# Autodesk Inventor assembly: #Spindexer
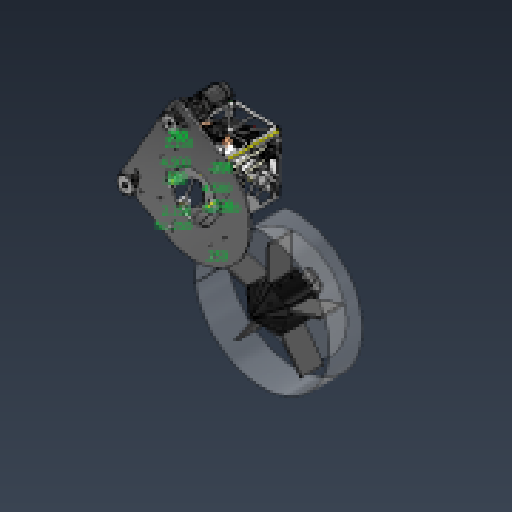
[picture p0: Inventor's stored thumbnail of the model, 512x512]
Saved by Autodesk Inventor 2026 (Build 300175050, 175E)
## iProperties
Created: 2026-02-05
Part Number: #Spindexer
Document SubType Name: Assembly
Designer: Owen L
Mass: 7775.4 g
Surface Area: 19734.6 cm^2
Volume: 5821.17 cm^3
Density: 1.33571 g/cm^3
Author: Owen L
## Documents named in this file (49)
- C:\Users\Jthib\Documents\GitHub\2026-Robot-Mechanical\Spindexer\#Spindexer.iam
- C:\Users\Jthib\Documents\GitHub\2026-Robot-Mechanical\Spindexer\3DPRINT,HUB.ipt
- C:\Users\Jthib\Documents\GitHub\2026-Robot-Mechanical\Spindexer\3DPRINT,HUB,CONE.ipt
- C:\Users\Jthib\Documents\GitHub\2026-Robot-Mechanical\Spindexer\PLATE,WALL.ipt
- C:\Users\Jthib\Documents\GitHub\2026-Robot-Mechanical\Spindexer\PLATE,BOTTOM.ipt
- C:\Users\Jthib\Documents\GitHub\2026-Robot-Mechanical\Spindexer\STOCK,HEX,SHAFT,HUB.ipt
- C:\Users\Jthib\Documents\GitHub\2026-Robot-Mechanical\Spindexer\PLATE,KICKER,OUTSIDE.ipt
- C:\Users\Jthib\Documents\GitHub\2026-Robot-Mechanical\Spindexer\3DPRINT,KICKER,RAMP.ipt
- C:\Users\Jthib\Documents\GitHub\2026-Robot-Mechanical\Spindexer\PLATE,KICKER,INSIDE.ipt
- C:\Users\Jthib\Documents\GitHub\2026-Robot-Mechanical\Spindexer\STOCK,HEX,SHAFT,KICKER,FRONT.ipt
- C:\Users\Jthib\Documents\GitHub\2026-Robot-Mechanical\Spindexer\STOCK,HEX,SHAFT,KICKER,BACK.ipt
- C:\Users\Jthib\Documents\GitHub\2026-Robot-Mechanical\#1_CAD Library\Power Transmission\Bearings\PURCHASED,HEX_BEARING.ipt
- C:\Users\Jthib\Documents\GitHub\2026-Robot-Mechanical\#1_CAD Library\Power Transmission\VersaPlanetary\GEARBOX,VERSAPLANETARY,SINGLE-STAGE,HEX-SHAFT,0.5IN.ipt
- C:\Users\Jthib\Documents\GitHub\2026-Robot-Mechanical\#1_CAD Library\Power Transmission\VersaPlanetary\ADAPTER,CIM-NEO,VERSAPLANETARY.ipt
- C:\Users\Jthib\Documents\GitHub\2026-Robot-Mechanical\#1_CAD Library\Motors\MOTOR,REV,NEO,V1-1.ipt
- C:\Users\Jthib\Documents\GitHub\2026-Robot-Mechanical\Spindexer\PLATE,NUT-BLOCK,3-LONG.ipt
- C:\Users\Jthib\Documents\GitHub\2026-Robot-Mechanical\Spindexer\PLATE,NUT-BLOCK,2-LONG.ipt
- C:\Users\Jthib\Documents\GitHub\2026-Robot-Mechanical\Spindexer\PLATE,NUT-BLOCK,1-LONG.ipt
- C:\Users\Jthib\Documents\GitHub\2026-Robot-Mechanical\#1_CAD Library\Electronics\CONTROLS,SPARK_MAX.ipt
- C:\Users\Jthib\Documents\GitHub\2026-Robot-Mechanical\Spindexer\3DPRINT,SPARK_MAX,MOUNT.ipt
- C:\Users\Jthib\Documents\GitHub\2026-Robot-Mechanical\Spindexer\PLATE,KICKER,BACK.ipt
- C:\Users\Jthib\Documents\GitHub\2026-Robot-Mechanical\Spindexer\PLATE,NUT-BLOCK,L-SHAPE.ipt
- C:\Users\Jthib\Documents\GitHub\2026-Robot-Mechanical\Spindexer\3DPRINTED,PULLEY,21T,9mm.ipt
- C:\Users\Jthib\Documents\GitHub\2026-Robot-Mechanical\#1_CAD Library\Power Transmission\Pulleys\PURCHASED,HTD5mm,24T,PULLEY.ipt
- C:\Users\Jthib\Documents\GitHub\2026-Robot-Mechanical\Spindexer\STANDIN,BELT,70T,HTD5mm.ipt
- C:\Users\Jthib\Documents\GitHub\2026-Robot-Mechanical\Spindexer\STANDIN,BELT,100T,HTD5mm.ipt
- C:\Users\Jthib\Documents\GitHub\2026-Robot-Mechanical\#1_CAD Library\Building Materials\Fasteners\Bolts\PURCHASED,10-32x0.5in,BUTTONHEAD,BOLT.ipt
- C:\Users\Jthib\Documents\GitHub\2026-Robot-Mechanical\#1_CAD Library\Building Materials\Fasteners\Nuts\PURCHASED,NYLOCK,10-32,NUT.ipt
- C:\Users\Jthib\Documents\GitHub\2026-Robot-Mechanical\#1_CAD Library\Building Materials\Fasteners\Bolts\PURCHASED,10-32x0.625in,BUTTONHEAD,BOLT.ipt
- C:\Users\Jthib\Documents\GitHub\2026-Robot-Mechanical\Spindexer\PLATE,NUT-BLOCK,SINGLE-L.ipt
- C:\Users\Jthib\Documents\GitHub\2026-Robot-Mechanical\Spindexer\PLATE,SHOOTER,MOUNT.ipt
- C:\Users\Jthib\Documents\GitHub\2026-Robot-Mechanical\Spindexer\#Spindexer\Design Accelerator\PLATE,TURRET,ENCODER,GEAR.ipt
- C:\Users\Jthib\Documents\GitHub\2026-Robot-Mechanical\Spindexer\#Spindexer\Design Accelerator\PLATE,TURRET,PINNION,GEAR.ipt
- C:\Users\Jthib\Documents\GitHub\2026-Robot-Mechanical\Spindexer\#Spindexer\Design Accelerator\PLATE,TURRET,MOTOR,MOUNT.ipt
- C:\Users\Jthib\Documents\GitHub\2026-Robot-Mechanical\#1_CAD Library\Electronics\CONTROLS,ENCODER,HEX_BORE.ipt
- C:\Users\Jthib\Documents\GitHub\2026-Robot-Mechanical\Spindexer\#Spindexer\Design Accelerator\STOCK,HEX,SHAFT,TURRET,DRIVE.ipt
- C:\Users\Jthib\Documents\GitHub\2026-Robot-Mechanical\Spindexer\#Spindexer\Design Accelerator\STOCK,HEX,SHAFT,TURRET,ENCODER.ipt
- C:\Users\Jthib\Documents\GitHub\2026-Robot-Mechanical\Spindexer\#Spindexer\Design Accelerator\3DPRINT,TURRET,HEX,SPACER.ipt
- C:\Users\Jthib\Documents\GitHub\2026-Robot-Mechanical\Spindexer\STOCK,CHURRO,HEX,TURRET,MOTOR-MOUNT,SPACER.ipt
- C:\Users\Jthib\Documents\GitHub\2026-Robot-Mechanical\#1_CAD Library\Building Materials\Fasteners\Bolts\PURCHASED,0.25-20x0.5in,BUTTONHEAD,BOLT.ipt
- C:\Users\Jthib\Documents\GitHub\2026-Robot-Mechanical\Spindexer\3DRPINT,FRONT-ROLLER,DRIVE-SPACER.ipt
- C:\Users\Jthib\Documents\GitHub\2026-Robot-Mechanical\Spindexer\CAST,SLAB-OF-FLOP.ipt
- C:\Users\Jthib\Documents\GitHub\2026-Robot-Mechanical\Spindexer\PURCHASED,20-1,90deg,MAX-PLANETARY.ipt
- C:\Users\Jthib\Documents\GitHub\2026-Robot-Mechanical\#1_CAD Library\Motors\MOTOR,NEO,V2.0.ipt
- C:\Users\Jthib\Documents\GitHub\2026-Robot-Mechanical\#1_CAD Library\Wheels\Compliant\PURCHASED,WHEEL,COMPLIANT,2.25in.ipt
- C:\Users\Jthib\Documents\GitHub\2026-Robot-Mechanical\Spindexer\MOTOR,VEX,FALCON,500.ipt
- C:\Users\Jthib\Documents\GitHub\2026-Robot-Mechanical\#1_CAD Library\Power Transmission\MaxPlanetary\PURCHASED,REV,MAX-PLANETARY,SINGLE-STAGE,FALCON-TO-HEX.ipt
- C:\Users\Jthib\Documents\GitHub\2026-Robot-Mechanical\#1_CAD Library\Building Materials\Fasteners\Bolts\PURCHASED,10-32x0.625in,FLATHEAD,BOLT.ipt
- C:\Users\Jthib\Documents\GitHub\2026-Robot-Mechanical\#1_CAD Library\Building Materials\Fasteners\Washers\PURCHASED,WASHER,10-32.ipt
## Components (176 placed, 48 different names)
1. 3DPRINT,HUB:1 — Mate:11, Mate:12, Mate:13, Mate:15, Mate:16, Mate:17, Flush:2, Mate:106, Mate:107, Mate:108, Mate:109, Mate:110, Mate:111, Mate:112, Mate:113, Mate:114, Mate:117, Mate:118, Mate:119, Mate:120
2. 3DPRINT,HUB,CONE:1 — Mate:11, Mate:12, Mate:13
3. PLATE,WALL:1 — Flush:8, Mate:42, Mate:43, Flush:24
4. PLATE,BOTTOM:1 — Mate:117, Mate:118, Mate:119, Flush:24, Mate:122
5. STOCK,HEX,SHAFT,HUB:1 — Mate:16, Mate:17, Flush:2, Mate:121
6. PLATE,KICKER,OUTSIDE:1 — Mate:22, Mate:23, Mate:24, Mate:25, Flush:3, Flush:4, Flush:8, Insert:1, Insert:4, Mate:34, Mate:35, Mate:42, Insert:9, Insert:10, Insert:13, Flush:12, Mate:43, Insert:23, Insert:24, Insert:34, Insert:35, Insert:39, Insert:40, Insert:41, Insert:42, Insert:43, Insert:44, Insert:45, Insert:46, Insert:47, Insert:48, Insert:49, Insert:50, Insert:79, Insert:80, Insert:81, Insert:82, Mate:59, Insert:83, Mate:62, Insert:87, Insert:93, Insert:94, Mate:65, Mate:138, Mate:139, Insert:213, Insert:214
7. 3DPRINT,KICKER,RAMP:1 — Mate:22, Mate:23, Mate:24
8. PLATE,KICKER,INSIDE:1 — Mate:25, Flush:3, Flush:4, Insert:2, Insert:3, Mate:39, Mate:40, Mate:41, Insert:14, Insert:21, Insert:22, Insert:31, Insert:32, Insert:33, Mate:48, Mate:52, Insert:61, Insert:65, Insert:66, Insert:67, Insert:68, Insert:69, Insert:70, Insert:71, Insert:72, Insert:73, Insert:74, Insert:75, Insert:76, Insert:77, Insert:78, Mate:60, Insert:84, Mate:61, Insert:90, Insert:210, Insert:211, Insert:212
9. STOCK,HEX,SHAFT,KICKER,FRONT:1 — Mate:34, Mate:45, Flush:15, Mate:128, Mate:129, Mate:130
10. STOCK,HEX,SHAFT,KICKER,BACK:1 — Mate:35, Mate:46, Mate:47, Flush:14, Mate:131, Mate:132, Mate:133
11. PURCHASED,HEX_BEARING:1 — Insert:1, Flush:15
12. PURCHASED,HEX_BEARING:2 — Insert:2, Mate:103, Mate:104
13. PURCHASED,HEX_BEARING:3 — Insert:3, Mate:63
14. PURCHASED,HEX_BEARING:4 — Insert:4, Flush:14
15. GEARBOX,VERSAPLANETARY,SINGLE-STAGE,HEX-SHAFT,0.5IN:1 — Mate:36, Mate:37, Mate:38, Mate:39, Mate:40, Mate:41, Mate:53
16. ADAPTER,CIM-NEO,VERSAPLANETARY:1 — Mate:36, Mate:37, Mate:38, Insert:5
17. MOTOR,REV,NEO,V1-1:1 — Insert:5
18. PLATE,NUT-BLOCK,3-LONG:1 — Mate:60, Insert:84
19. PLATE,NUT-BLOCK,3-LONG:2 — Insert:9, Insert:10
20. PLATE,NUT-BLOCK,3-LONG:3 — Mate:59, Insert:83
21. PLATE,NUT-BLOCK,1-LONG:1 — Insert:13, Flush:11, Flush:12
22. PLATE,NUT-BLOCK,1-LONG:2 — Insert:14, Flush:11
23. PLATE,NUT-BLOCK,3-LONG:4 — Mate:66, Insert:210
24. PLATE,NUT-BLOCK,3-LONG:5 — Insert:93, Insert:94, Mate:67
25. CONTROLS,SPARK_MAX:1 — Mate:125, Mate:126, Mate:127
26. 3DPRINT,SPARK_MAX,MOUNT:1 — Insert:149, Mate:124, Mate:126, Mate:127
27. PLATE,KICKER,BACK:1 — Mate:44, Insert:25, Insert:26, Insert:27, Insert:28, Insert:51, Insert:52, Insert:53, Insert:54, Insert:55, Insert:59, Insert:60, Insert:85, Insert:86, Insert:88, Insert:89, Insert:149, Mate:124, Mate:125, Insert:229, Insert:230
28. PLATE,NUT-BLOCK,2-LONG:2 — Insert:21, Insert:22, Mate:44, Insert:26
29. PLATE,NUT-BLOCK,2-LONG:3 — Insert:23, Insert:24, Insert:25
30. PLATE,NUT-BLOCK,3-LONG:6 — Insert:27, Insert:28
31. PLATE,NUT-BLOCK,3-LONG:8 — Insert:31, Insert:32
32. PLATE,NUT-BLOCK,L-SHAPE:1 — Insert:33
33. PLATE,NUT-BLOCK,L-SHAPE:2 — Insert:34
34. 3DPRINTED,PULLEY,21T,9mm:1 — Mate:46, Mate:55, Mate:58, Mate:64, Flush:16
35. 3DPRINTED,PULLEY,21T,9mm:2 — Mate:45, Mate:54, Flush:16
36. PURCHASED,HEX_BEARING:5 — Mate:52, Mate:53
37. PURCHASED,HTD5mm,24T,PULLEY:1 — Mate:47, Flush:13, Mate:57, Mate:63, Mate:64
38. PURCHASED,HTD5mm,24T,PULLEY:2 — Mate:48, Flush:13, Mate:56
39. STANDIN,BELT,70T,HTD5mm:1 — Mate:56, Mate:57
40. STANDIN,BELT,100T,HTD5mm:1 — Mate:54, Mate:55, Mate:58
41. PURCHASED,10-32x0.5in,BUTTONHEAD,BOLT:1 — Insert:48
42. PURCHASED,NYLOCK,10-32,NUT:1 — Insert:81
43. PURCHASED,10-32x0.625in,BUTTONHEAD,BOLT:1 — Insert:35
44. PURCHASED,10-32x0.625in,BUTTONHEAD,BOLT:5 — Insert:39
45. PURCHASED,10-32x0.625in,BUTTONHEAD,BOLT:6 — Insert:40
46. PURCHASED,10-32x0.625in,BUTTONHEAD,BOLT:7 — Insert:41
47. PURCHASED,10-32x0.625in,BUTTONHEAD,BOLT:8 — Insert:42
48. PURCHASED,10-32x0.625in,BUTTONHEAD,BOLT:9 — Insert:43
49. PURCHASED,10-32x0.625in,BUTTONHEAD,BOLT:10 — Insert:44
50. PURCHASED,10-32x0.625in,BUTTONHEAD,BOLT:11 — Insert:45
51. PURCHASED,10-32x0.625in,BUTTONHEAD,BOLT:12 — Insert:46
52. PURCHASED,10-32x0.625in,BUTTONHEAD,BOLT:13 — Insert:47
53. PURCHASED,10-32x0.625in,BUTTONHEAD,BOLT:14 — Insert:51
54. PURCHASED,10-32x0.625in,BUTTONHEAD,BOLT:15 — Insert:52
55. PURCHASED,10-32x0.625in,BUTTONHEAD,BOLT:16 — Insert:53
56. PURCHASED,10-32x0.625in,BUTTONHEAD,BOLT:17 — Insert:54
57. PURCHASED,10-32x0.625in,BUTTONHEAD,BOLT:18 — Insert:55
58. PURCHASED,10-32x0.5in,BUTTONHEAD,BOLT:2 — Insert:49
59. PURCHASED,10-32x0.5in,BUTTONHEAD,BOLT:3 — Insert:50
60. PURCHASED,10-32x0.625in,BUTTONHEAD,BOLT:19 — Insert:59
61. PURCHASED,10-32x0.625in,BUTTONHEAD,BOLT:20 — Insert:89
62. PURCHASED,10-32x0.625in,BUTTONHEAD,BOLT:21 — Insert:87
63. PURCHASED,10-32x0.625in,BUTTONHEAD,BOLT:22 — Insert:60
64. PURCHASED,10-32x0.625in,BUTTONHEAD,BOLT:23 — Insert:88
65. PURCHASED,10-32x0.625in,BUTTONHEAD,BOLT:24 — Insert:61
66. PURCHASED,10-32x0.625in,BUTTONHEAD,BOLT:28 — Insert:65
67. PURCHASED,10-32x0.625in,BUTTONHEAD,BOLT:29 — Insert:66
68. PURCHASED,10-32x0.625in,BUTTONHEAD,BOLT:30 — Insert:67
69. PURCHASED,10-32x0.625in,BUTTONHEAD,BOLT:31 — Insert:68
70. PURCHASED,10-32x0.625in,BUTTONHEAD,BOLT:32 — Insert:69
71. PURCHASED,10-32x0.625in,BUTTONHEAD,BOLT:33 — Insert:70
72. PURCHASED,10-32x0.625in,BUTTONHEAD,BOLT:34 — Insert:73
73. PURCHASED,10-32x0.625in,BUTTONHEAD,BOLT:35 — Insert:72
74. PURCHASED,10-32x0.625in,BUTTONHEAD,BOLT:36 — Insert:71
75. PURCHASED,10-32x0.5in,BUTTONHEAD,BOLT:4 — Insert:74
76. PURCHASED,10-32x0.5in,BUTTONHEAD,BOLT:5 — Insert:76
77. PURCHASED,10-32x0.5in,BUTTONHEAD,BOLT:6 — Insert:75
78. PURCHASED,10-32x0.5in,BUTTONHEAD,BOLT:7 — Insert:77
79. PURCHASED,10-32x0.5in,BUTTONHEAD,BOLT:8 — Insert:78
80. PURCHASED,10-32x0.5in,BUTTONHEAD,BOLT:9 — Insert:79
81. PURCHASED,10-32x0.5in,BUTTONHEAD,BOLT:10 — Insert:80
82. PURCHASED,NYLOCK,10-32,NUT:2 — Insert:82
83. PLATE,NUT-BLOCK,SINGLE-L:1 — Insert:85, Mate:61
84. PLATE,NUT-BLOCK,SINGLE-L:2 — Insert:86, Mate:62
85. PURCHASED,10-32x0.625in,BUTTONHEAD,BOLT:37 — Insert:90
86. PLATE,SHOOTER,MOUNT:1 — Mate:65, Mate:66, Mate:67, Mate:82, Mate:95, Mate:100, Insert:142, Insert:143, Insert:144, Insert:145, Insert:146, Insert:147, Insert:150, Insert:151, Insert:152, Insert:153, Insert:154, Insert:158, Insert:159, Insert:160, Insert:164, Insert:165, Insert:166, Insert:168, Insert:169, Insert:170, Mate:150, Mate:151, Insert:185, Insert:186, Insert:187, Insert:188, Insert:221, Insert:222, Insert:223, Insert:224, Insert:225, Insert:226, Insert:227, Insert:228, Insert:231, Insert:233, Insert:235, Insert:237
87. PLATE,TURRET,ENCODER,GEAR:1 — Mate:102, Mate:143, Flush:26
88. PLATE,TURRET,PINNION,GEAR:1 — Mate:86, Flush:25, Mate:140, Mate:141
89. PURCHASED,HEX_BEARING:6 — Mate:83, Mate:86, Mate:93, Insert:154
90. PURCHASED,HEX_BEARING:7 — Mate:94, Mate:96, Insert:153, Mate:145
91. PLATE,TURRET,MOTOR,MOUNT:1 — Mate:100, Insert:155, Insert:156, Insert:157, Insert:161, Insert:162, Insert:163, Insert:174, Insert:175, Insert:176, Insert:177, Mate:147, Insert:178, Mate:148
92. CONTROLS,ENCODER,HEX_BORE:1 — Mate:95, Mate:96, Insert:236, Insert:238
93. CONTROLS,ENCODER,HEX_BORE:2 — Mate:82, Mate:83, Insert:232, Insert:234
94. STOCK,HEX,SHAFT,TURRET,DRIVE:1 — Flush:25, Mate:140, Mate:142, Insert:215
95. STOCK,HEX,SHAFT,TURRET,ENCODER:1 — Mate:143, Flush:26, Mate:144, Insert:216, Insert:217
96. 3DPRINT,TURRET,HEX,SPACER:1 — Mate:94, Mate:102, Mate:144, Mate:145
97. 3DPRINT,TURRET,HEX,SPACER:2 — Mate:93, Mate:141, Mate:142
98. PURCHASED,10-32x0.625in,BUTTONHEAD,BOLT:44 — Mate:150, Insert:231
99. PURCHASED,10-32x0.625in,BUTTONHEAD,BOLT:45 — Insert:233
100. PURCHASED,NYLOCK,10-32,NUT:5 — Insert:234
101. PURCHASED,NYLOCK,10-32,NUT:6 — Insert:232
102. STOCK,CHURRO,HEX,TURRET,MOTOR-MOUNT,SPACER:1 — Insert:150
103. STOCK,CHURRO,HEX,TURRET,MOTOR-MOUNT,SPACER:2 — Insert:152, Insert:157
104. STOCK,CHURRO,HEX,TURRET,MOTOR-MOUNT,SPACER:3 — Insert:151, Insert:156
105. STOCK,CHURRO,HEX,TURRET,MOTOR-MOUNT,SPACER:4 — Insert:164, Mate:146
106. PURCHASED,0.25-20x0.5in,BUTTONHEAD,BOLT:4 — Insert:158
107. 3DRPINT,FRONT-ROLLER,DRIVE-SPACER:1 — Mate:103, Mate:104
108. PURCHASED,10-32x0.625in,BUTTONHEAD,BOLT:46 — Mate:151, Insert:237
109. PURCHASED,10-32x0.625in,BUTTONHEAD,BOLT:47 — Insert:235
110. PURCHASED,NYLOCK,10-32,NUT:7 — Insert:238
111. PURCHASED,NYLOCK,10-32,NUT:8 — Insert:236
112. CAST,SLAB-OF-FLOP:1 — Mate:106, Mate:107
113. CAST,SLAB-OF-FLOP:2 — Mate:108, Mate:109
114. CAST,SLAB-OF-FLOP:3 — Mate:110, Mate:111
115. CAST,SLAB-OF-FLOP:4 — Mate:112, Mate:113
116. CAST,SLAB-OF-FLOP:5 — Mate:114, Mate:120
117. PURCHASED,10-32x0.625in,BUTTONHEAD,BOLT:52 — Insert:142
118. PURCHASED,10-32x0.625in,BUTTONHEAD,BOLT:53 — Insert:143
119. PURCHASED,10-32x0.625in,BUTTONHEAD,BOLT:54 — Insert:144
120. PURCHASED,10-32x0.625in,BUTTONHEAD,BOLT:55 — Insert:145
121. PURCHASED,10-32x0.625in,BUTTONHEAD,BOLT:56 — Insert:146
122. PURCHASED,10-32x0.625in,BUTTONHEAD,BOLT:57 — Insert:147
123. PURCHASED,20-1,90deg,MAX-PLANETARY:1 — Mate:121, Mate:122, Insert:148, Mate:123
124. MOTOR,NEO,V2.0:1 — Insert:148, Mate:123
125. PURCHASED,WHEEL,COMPLIANT,2.25in:1 — Mate:128, Mate:136, Mate:137
126. PURCHASED,WHEEL,COMPLIANT,2.25in:2 — Mate:129, Mate:137
127. PURCHASED,WHEEL,COMPLIANT,2.25in:3 — Mate:130, Mate:136, Mate:138
128. PURCHASED,WHEEL,COMPLIANT,2.25in:4 — Mate:133, Mate:134
129. PURCHASED,WHEEL,COMPLIANT,2.25in:5 — Mate:131, Mate:134, Mate:135
130. PURCHASED,WHEEL,COMPLIANT,2.25in:6 — Mate:132, Mate:135, Mate:139
131. PURCHASED,HEX_BEARING:8 — Insert:155
132. PURCHASED,0.25-20x0.5in,BUTTONHEAD,BOLT:5 — Insert:160
133. PURCHASED,0.25-20x0.5in,BUTTONHEAD,BOLT:6 — Insert:159
134. PURCHASED,0.25-20x0.5in,BUTTONHEAD,BOLT:7 — Insert:161
135. PURCHASED,0.25-20x0.5in,BUTTONHEAD,BOLT:8 — Insert:162
136. PURCHASED,0.25-20x0.5in,BUTTONHEAD,BOLT:9 — Insert:163
137. PLATE,TURRET,MOTOR,MOUNT:2 — Insert:167, Mate:146, Insert:171, Insert:172, Insert:173, Insert:180
138. STOCK,CHURRO,HEX,TURRET,MOTOR-MOUNT,SPACER:5 — Insert:165, Insert:167
139. STOCK,CHURRO,HEX,TURRET,MOTOR-MOUNT,SPACER:6 — Insert:166
140. PURCHASED,0.25-20x0.5in,BUTTONHEAD,BOLT:10 — Insert:168
141. PURCHASED,0.25-20x0.5in,BUTTONHEAD,BOLT:11 — Insert:169
142. PURCHASED,0.25-20x0.5in,BUTTONHEAD,BOLT:12 — Insert:170
143. PURCHASED,0.25-20x0.5in,BUTTONHEAD,BOLT:13 — Insert:171
144. PURCHASED,0.25-20x0.5in,BUTTONHEAD,BOLT:14 — Insert:172
145. PURCHASED,0.25-20x0.5in,BUTTONHEAD,BOLT:15 — Insert:173
146. PURCHASED,10-32x0.625in,BUTTONHEAD,BOLT:58 — Insert:177
147. PURCHASED,10-32x0.625in,BUTTONHEAD,BOLT:59 — Insert:176
148. PURCHASED,10-32x0.625in,BUTTONHEAD,BOLT:60 — Insert:175
149. PURCHASED,10-32x0.625in,BUTTONHEAD,BOLT:61 — Insert:174
150. MOTOR,VEX,FALCON,500:1 — Insert:179, Mate:149
151. PURCHASED,REV,MAX-PLANETARY,SINGLE-STAGE,FALCON-TO-HEX:1 — Mate:147, Insert:178, Mate:148, Insert:179, Mate:149
152. PURCHASED,HEX_BEARING:9 — Insert:180
153. PURCHASED,10-32x0.625in,FLATHEAD,BOLT:1 — Insert:185
154. PURCHASED,10-32x0.625in,FLATHEAD,BOLT:2 — Insert:186
155. PURCHASED,10-32x0.625in,FLATHEAD,BOLT:3 — Insert:187
156. PURCHASED,10-32x0.625in,FLATHEAD,BOLT:4 — Insert:188
157. PURCHASED,10-32x0.625in,FLATHEAD,BOLT:5 — Insert:211
158. PURCHASED,10-32x0.625in,FLATHEAD,BOLT:6 — Insert:212
159. PURCHASED,10-32x0.625in,FLATHEAD,BOLT:7 — Insert:214
160. PURCHASED,10-32x0.625in,FLATHEAD,BOLT:8 — Insert:213
161. PURCHASED,WASHER,10-32:11 — Insert:215, Insert:218
162. PURCHASED,WASHER,10-32:12 — Insert:217, Insert:220
163. PURCHASED,WASHER,10-32:13 — Insert:216, Insert:219
164. PURCHASED,10-32x0.625in,BUTTONHEAD,BOLT:62 — Insert:218
165. PURCHASED,10-32x0.625in,BUTTONHEAD,BOLT:63 — Insert:219
166. PURCHASED,10-32x0.625in,BUTTONHEAD,BOLT:64 — Insert:220
167. PURCHASED,10-32x0.5in,BUTTONHEAD,BOLT:11 — Insert:221
168. PURCHASED,10-32x0.5in,BUTTONHEAD,BOLT:12 — Insert:222
169. PURCHASED,10-32x0.5in,BUTTONHEAD,BOLT:13 — Insert:223
170. PURCHASED,10-32x0.5in,BUTTONHEAD,BOLT:14 — Insert:224
171. PURCHASED,10-32x0.5in,BUTTONHEAD,BOLT:15 — Insert:225
172. PURCHASED,10-32x0.5in,BUTTONHEAD,BOLT:16 — Insert:226
173. PURCHASED,10-32x0.5in,BUTTONHEAD,BOLT:17 — Insert:227
174. PURCHASED,10-32x0.5in,BUTTONHEAD,BOLT:18 — Insert:228
175. PURCHASED,10-32x0.625in,BUTTONHEAD,BOLT:65 — Insert:229
176. PURCHASED,10-32x0.625in,BUTTONHEAD,BOLT:66 — Insert:230
## Relationships (251: Insert 142, Mate 96, Flush 13)
- Mate:11: 3DPRINT,HUB:1 ↔ 3DPRINT,HUB,CONE:1
- Mate:12: 3DPRINT,HUB:1 ↔ 3DPRINT,HUB,CONE:1
- Mate:13: 3DPRINT,HUB:1 ↔ 3DPRINT,HUB,CONE:1
- Mate:15: 3DPRINT,HUB:1
- Mate:16: 3DPRINT,HUB:1 ↔ STOCK,HEX,SHAFT,HUB:1
- Mate:17: 3DPRINT,HUB:1 ↔ STOCK,HEX,SHAFT,HUB:1
- Flush:2 (-12.7 mm): 3DPRINT,HUB:1 ↔ STOCK,HEX,SHAFT,HUB:1
- Mate:22: PLATE,KICKER,OUTSIDE:1 ↔ 3DPRINT,KICKER,RAMP:1
- Mate:23: PLATE,KICKER,OUTSIDE:1 ↔ 3DPRINT,KICKER,RAMP:1
- Mate:24: PLATE,KICKER,OUTSIDE:1 ↔ 3DPRINT,KICKER,RAMP:1
- Mate:25 (158.75 mm): PLATE,KICKER,OUTSIDE:1 ↔ PLATE,KICKER,INSIDE:1
- Flush:3: PLATE,KICKER,OUTSIDE:1 ↔ PLATE,KICKER,INSIDE:1
- Flush:4: PLATE,KICKER,OUTSIDE:1 ↔ PLATE,KICKER,INSIDE:1
- Flush:8: PLATE,WALL:1 ↔ PLATE,KICKER,OUTSIDE:1
- Insert:1: PLATE,KICKER,OUTSIDE:1 ↔ PURCHASED,HEX_BEARING:1
- Insert:2: PLATE,KICKER,INSIDE:1 ↔ PURCHASED,HEX_BEARING:2
- Insert:3: PLATE,KICKER,INSIDE:1 ↔ PURCHASED,HEX_BEARING:3
- Insert:4: PLATE,KICKER,OUTSIDE:1 ↔ PURCHASED,HEX_BEARING:4
- Mate:34: PLATE,KICKER,OUTSIDE:1 ↔ STOCK,HEX,SHAFT,KICKER,FRONT:1
- Mate:35: PLATE,KICKER,OUTSIDE:1 ↔ STOCK,HEX,SHAFT,KICKER,BACK:1
- Mate:36: GEARBOX,VERSAPLANETARY,SINGLE-STAGE,HEX-SHAFT,0.5IN:1 ↔ ADAPTER,CIM-NEO,VERSAPLANETARY:1
- Mate:37: GEARBOX,VERSAPLANETARY,SINGLE-STAGE,HEX-SHAFT,0.5IN:1 ↔ ADAPTER,CIM-NEO,VERSAPLANETARY:1
- Mate:38: GEARBOX,VERSAPLANETARY,SINGLE-STAGE,HEX-SHAFT,0.5IN:1 ↔ ADAPTER,CIM-NEO,VERSAPLANETARY:1
- Insert:5: ADAPTER,CIM-NEO,VERSAPLANETARY:1 ↔ MOTOR,REV,NEO,V1-1:1
- Mate:39: PLATE,KICKER,INSIDE:1 ↔ GEARBOX,VERSAPLANETARY,SINGLE-STAGE,HEX-SHAFT,0.5IN:1
- Mate:40: PLATE,KICKER,INSIDE:1 ↔ GEARBOX,VERSAPLANETARY,SINGLE-STAGE,HEX-SHAFT,0.5IN:1
- Mate:41: PLATE,KICKER,INSIDE:1 ↔ GEARBOX,VERSAPLANETARY,SINGLE-STAGE,HEX-SHAFT,0.5IN:1
- Mate:42: PLATE,WALL:1 ↔ PLATE,KICKER,OUTSIDE:1
- Insert:9: PLATE,KICKER,OUTSIDE:1 ↔ PLATE,NUT-BLOCK,3-LONG:2
- Insert:10: PLATE,KICKER,OUTSIDE:1 ↔ PLATE,NUT-BLOCK,3-LONG:2
- Insert:13: PLATE,KICKER,OUTSIDE:1 ↔ PLATE,NUT-BLOCK,1-LONG:1
- Insert:14: PLATE,KICKER,INSIDE:1 ↔ PLATE,NUT-BLOCK,1-LONG:2
- Flush:11: PLATE,NUT-BLOCK,1-LONG:1 ↔ PLATE,NUT-BLOCK,1-LONG:2
- Flush:12: PLATE,KICKER,OUTSIDE:1 ↔ PLATE,NUT-BLOCK,1-LONG:1
- Mate:43 (-25.4 mm): PLATE,WALL:1 ↔ PLATE,KICKER,OUTSIDE:1
- Insert:21: PLATE,KICKER,INSIDE:1 ↔ PLATE,NUT-BLOCK,2-LONG:2
- Insert:22: PLATE,KICKER,INSIDE:1 ↔ PLATE,NUT-BLOCK,2-LONG:2
- Insert:23: PLATE,KICKER,OUTSIDE:1 ↔ PLATE,NUT-BLOCK,2-LONG:3
- Insert:24: PLATE,KICKER,OUTSIDE:1 ↔ PLATE,NUT-BLOCK,2-LONG:3
- Mate:44: PLATE,KICKER,BACK:1 ↔ PLATE,NUT-BLOCK,2-LONG:2
- Insert:25: PLATE,KICKER,BACK:1 ↔ PLATE,NUT-BLOCK,2-LONG:3
- Insert:26: PLATE,KICKER,BACK:1 ↔ PLATE,NUT-BLOCK,2-LONG:2
- Insert:27: PLATE,KICKER,BACK:1 ↔ PLATE,NUT-BLOCK,3-LONG:6
- Insert:28: PLATE,KICKER,BACK:1 ↔ PLATE,NUT-BLOCK,3-LONG:6
- Insert:31: PLATE,KICKER,INSIDE:1 ↔ PLATE,NUT-BLOCK,3-LONG:8
- Insert:32: PLATE,KICKER,INSIDE:1 ↔ PLATE,NUT-BLOCK,3-LONG:8
- Insert:33: PLATE,KICKER,INSIDE:1 ↔ PLATE,NUT-BLOCK,L-SHAPE:1
- Insert:34: PLATE,KICKER,OUTSIDE:1 ↔ PLATE,NUT-BLOCK,L-SHAPE:2
- Mate:45: STOCK,HEX,SHAFT,KICKER,FRONT:1 ↔ 3DPRINTED,PULLEY,21T,9mm:2
- Mate:46: STOCK,HEX,SHAFT,KICKER,BACK:1 ↔ 3DPRINTED,PULLEY,21T,9mm:1
- Mate:47: STOCK,HEX,SHAFT,KICKER,BACK:1 ↔ PURCHASED,HTD5mm,24T,PULLEY:1
- Mate:48: PLATE,KICKER,INSIDE:1 ↔ PURCHASED,HTD5mm,24T,PULLEY:2
- Flush:13: PURCHASED,HTD5mm,24T,PULLEY:1 ↔ PURCHASED,HTD5mm,24T,PULLEY:2
- Flush:14: STOCK,HEX,SHAFT,KICKER,BACK:1 ↔ PURCHASED,HEX_BEARING:4
- Flush:15: STOCK,HEX,SHAFT,KICKER,FRONT:1 ↔ PURCHASED,HEX_BEARING:1
- Mate:52: PLATE,KICKER,INSIDE:1 ↔ PURCHASED,HEX_BEARING:5
- Mate:53: GEARBOX,VERSAPLANETARY,SINGLE-STAGE,HEX-SHAFT,0.5IN:1 ↔ PURCHASED,HEX_BEARING:5
- Mate:54: 3DPRINTED,PULLEY,21T,9mm:2 ↔ STANDIN,BELT,100T,HTD5mm:1
- Mate:55: 3DPRINTED,PULLEY,21T,9mm:1 ↔ STANDIN,BELT,100T,HTD5mm:1
- Mate:56: PURCHASED,HTD5mm,24T,PULLEY:2 ↔ STANDIN,BELT,70T,HTD5mm:1
- Mate:57: PURCHASED,HTD5mm,24T,PULLEY:1 ↔ STANDIN,BELT,70T,HTD5mm:1
- Mate:58: 3DPRINTED,PULLEY,21T,9mm:1 ↔ STANDIN,BELT,100T,HTD5mm:1
- Insert:35: PLATE,KICKER,OUTSIDE:1 ↔ PURCHASED,10-32x0.625in,BUTTONHEAD,BOLT:1
- Insert:39: PLATE,KICKER,OUTSIDE:1 ↔ PURCHASED,10-32x0.625in,BUTTONHEAD,BOLT:5
- Insert:40: PLATE,KICKER,OUTSIDE:1 ↔ PURCHASED,10-32x0.625in,BUTTONHEAD,BOLT:6
- Insert:41: PLATE,KICKER,OUTSIDE:1 ↔ PURCHASED,10-32x0.625in,BUTTONHEAD,BOLT:7
- Insert:42: PLATE,KICKER,OUTSIDE:1 ↔ PURCHASED,10-32x0.625in,BUTTONHEAD,BOLT:8
- Insert:43: PLATE,KICKER,OUTSIDE:1 ↔ PURCHASED,10-32x0.625in,BUTTONHEAD,BOLT:9
- Insert:44: PLATE,KICKER,OUTSIDE:1 ↔ PURCHASED,10-32x0.625in,BUTTONHEAD,BOLT:10
- Insert:45: PLATE,KICKER,OUTSIDE:1 ↔ PURCHASED,10-32x0.625in,BUTTONHEAD,BOLT:11
- Insert:46: PLATE,KICKER,OUTSIDE:1 ↔ PURCHASED,10-32x0.625in,BUTTONHEAD,BOLT:12
- Insert:47: PLATE,KICKER,OUTSIDE:1 ↔ PURCHASED,10-32x0.625in,BUTTONHEAD,BOLT:13
- Insert:48: PLATE,KICKER,OUTSIDE:1 ↔ PURCHASED,10-32x0.5in,BUTTONHEAD,BOLT:1
- Insert:49: PLATE,KICKER,OUTSIDE:1 ↔ PURCHASED,10-32x0.5in,BUTTONHEAD,BOLT:2
- Insert:50: PLATE,KICKER,OUTSIDE:1 ↔ PURCHASED,10-32x0.5in,BUTTONHEAD,BOLT:3
- Insert:51: PLATE,KICKER,BACK:1 ↔ PURCHASED,10-32x0.625in,BUTTONHEAD,BOLT:14
- Insert:52: PLATE,KICKER,BACK:1 ↔ PURCHASED,10-32x0.625in,BUTTONHEAD,BOLT:15
- Insert:53: PLATE,KICKER,BACK:1 ↔ PURCHASED,10-32x0.625in,BUTTONHEAD,BOLT:16
- Insert:54: PLATE,KICKER,BACK:1 ↔ PURCHASED,10-32x0.625in,BUTTONHEAD,BOLT:17
- Insert:55: PLATE,KICKER,BACK:1 ↔ PURCHASED,10-32x0.625in,BUTTONHEAD,BOLT:18
- Insert:59: PLATE,KICKER,BACK:1 ↔ PURCHASED,10-32x0.625in,BUTTONHEAD,BOLT:19
- Insert:60: PLATE,KICKER,BACK:1 ↔ PURCHASED,10-32x0.625in,BUTTONHEAD,BOLT:22
- Insert:61: PLATE,KICKER,INSIDE:1 ↔ PURCHASED,10-32x0.625in,BUTTONHEAD,BOLT:24
- Insert:65: PLATE,KICKER,INSIDE:1 ↔ PURCHASED,10-32x0.625in,BUTTONHEAD,BOLT:28
- Insert:66: PLATE,KICKER,INSIDE:1 ↔ PURCHASED,10-32x0.625in,BUTTONHEAD,BOLT:29
- Insert:67: PLATE,KICKER,INSIDE:1 ↔ PURCHASED,10-32x0.625in,BUTTONHEAD,BOLT:30
- Insert:68: PLATE,KICKER,INSIDE:1 ↔ PURCHASED,10-32x0.625in,BUTTONHEAD,BOLT:31
- Insert:69: PLATE,KICKER,INSIDE:1 ↔ PURCHASED,10-32x0.625in,BUTTONHEAD,BOLT:32
- Insert:70: PLATE,KICKER,INSIDE:1 ↔ PURCHASED,10-32x0.625in,BUTTONHEAD,BOLT:33
- Insert:71: PLATE,KICKER,INSIDE:1 ↔ PURCHASED,10-32x0.625in,BUTTONHEAD,BOLT:36
- Insert:72: PLATE,KICKER,INSIDE:1 ↔ PURCHASED,10-32x0.625in,BUTTONHEAD,BOLT:35
- Insert:73: PLATE,KICKER,INSIDE:1 ↔ PURCHASED,10-32x0.625in,BUTTONHEAD,BOLT:34
- Insert:74: PLATE,KICKER,INSIDE:1 ↔ PURCHASED,10-32x0.5in,BUTTONHEAD,BOLT:4
- Insert:75: PLATE,KICKER,INSIDE:1 ↔ PURCHASED,10-32x0.5in,BUTTONHEAD,BOLT:6
- Insert:76: PLATE,KICKER,INSIDE:1 ↔ PURCHASED,10-32x0.5in,BUTTONHEAD,BOLT:5
- Insert:77: PLATE,KICKER,INSIDE:1 ↔ PURCHASED,10-32x0.5in,BUTTONHEAD,BOLT:7
- Insert:78: PLATE,KICKER,INSIDE:1 ↔ PURCHASED,10-32x0.5in,BUTTONHEAD,BOLT:8
- Insert:79: PLATE,KICKER,OUTSIDE:1 ↔ PURCHASED,10-32x0.5in,BUTTONHEAD,BOLT:9
- Insert:80: PLATE,KICKER,OUTSIDE:1 ↔ PURCHASED,10-32x0.5in,BUTTONHEAD,BOLT:10
- Insert:81: PLATE,KICKER,OUTSIDE:1 ↔ PURCHASED,NYLOCK,10-32,NUT:1
- Insert:82: PLATE,KICKER,OUTSIDE:1 ↔ PURCHASED,NYLOCK,10-32,NUT:2
- Mate:59: PLATE,KICKER,OUTSIDE:1 ↔ PLATE,NUT-BLOCK,3-LONG:3
- Insert:83: PLATE,KICKER,OUTSIDE:1 ↔ PLATE,NUT-BLOCK,3-LONG:3
- Mate:60: PLATE,KICKER,INSIDE:1 ↔ PLATE,NUT-BLOCK,3-LONG:1
- Insert:84: PLATE,KICKER,INSIDE:1 ↔ PLATE,NUT-BLOCK,3-LONG:1
- Insert:85: PLATE,KICKER,BACK:1 ↔ PLATE,NUT-BLOCK,SINGLE-L:1
- Mate:61: PLATE,KICKER,INSIDE:1 ↔ PLATE,NUT-BLOCK,SINGLE-L:1
- Insert:86: PLATE,KICKER,BACK:1 ↔ PLATE,NUT-BLOCK,SINGLE-L:2
- Mate:62: PLATE,KICKER,OUTSIDE:1 ↔ PLATE,NUT-BLOCK,SINGLE-L:2
- Insert:87: PLATE,KICKER,OUTSIDE:1 ↔ PURCHASED,10-32x0.625in,BUTTONHEAD,BOLT:21
- Insert:88: PLATE,KICKER,BACK:1 ↔ PURCHASED,10-32x0.625in,BUTTONHEAD,BOLT:23
- Insert:89: PLATE,KICKER,BACK:1 ↔ PURCHASED,10-32x0.625in,BUTTONHEAD,BOLT:20
- Insert:90: PLATE,KICKER,INSIDE:1 ↔ PURCHASED,10-32x0.625in,BUTTONHEAD,BOLT:37
- Mate:63: PURCHASED,HEX_BEARING:3 ↔ PURCHASED,HTD5mm,24T,PULLEY:1
- Mate:64: 3DPRINTED,PULLEY,21T,9mm:1 ↔ PURCHASED,HTD5mm,24T,PULLEY:1
- Flush:16: 3DPRINTED,PULLEY,21T,9mm:1 ↔ 3DPRINTED,PULLEY,21T,9mm:2
- Insert:93: PLATE,KICKER,OUTSIDE:1 ↔ PLATE,NUT-BLOCK,3-LONG:5
- Insert:94: PLATE,KICKER,OUTSIDE:1 ↔ PLATE,NUT-BLOCK,3-LONG:5
- Mate:65: PLATE,KICKER,OUTSIDE:1 ↔ PLATE,SHOOTER,MOUNT:1
- Mate:66: PLATE,NUT-BLOCK,3-LONG:4 ↔ PLATE,SHOOTER,MOUNT:1
- Mate:67: PLATE,NUT-BLOCK,3-LONG:5 ↔ PLATE,SHOOTER,MOUNT:1
- Mate:82: PLATE,SHOOTER,MOUNT:1 ↔ CONTROLS,ENCODER,HEX_BORE:2
- Mate:83: PURCHASED,HEX_BEARING:6 ↔ CONTROLS,ENCODER,HEX_BORE:2
- Mate:86: PLATE,TURRET,PINNION,GEAR:1 ↔ PURCHASED,HEX_BEARING:6
- Mate:93: PURCHASED,HEX_BEARING:6 ↔ 3DPRINT,TURRET,HEX,SPACER:2
- Mate:94: PURCHASED,HEX_BEARING:7 ↔ 3DPRINT,TURRET,HEX,SPACER:1
- Mate:95: PLATE,SHOOTER,MOUNT:1 ↔ CONTROLS,ENCODER,HEX_BORE:1
- Mate:96: PURCHASED,HEX_BEARING:7 ↔ CONTROLS,ENCODER,HEX_BORE:1
- Mate:100 (19.05 mm): PLATE,SHOOTER,MOUNT:1 ↔ PLATE,TURRET,MOTOR,MOUNT:1
- Mate:102: PLATE,TURRET,ENCODER,GEAR:1 ↔ 3DPRINT,TURRET,HEX,SPACER:1
- Mate:103: PURCHASED,HEX_BEARING:2 ↔ 3DRPINT,FRONT-ROLLER,DRIVE-SPACER:1
- Mate:104: PURCHASED,HEX_BEARING:2 ↔ 3DRPINT,FRONT-ROLLER,DRIVE-SPACER:1
- Mate:106: 3DPRINT,HUB:1 ↔ CAST,SLAB-OF-FLOP:1
- Mate:107: 3DPRINT,HUB:1 ↔ CAST,SLAB-OF-FLOP:1
- Mate:108: 3DPRINT,HUB:1 ↔ CAST,SLAB-OF-FLOP:2
- Mate:109: 3DPRINT,HUB:1 ↔ CAST,SLAB-OF-FLOP:2
- Mate:110: 3DPRINT,HUB:1 ↔ CAST,SLAB-OF-FLOP:3
- Mate:111: 3DPRINT,HUB:1 ↔ CAST,SLAB-OF-FLOP:3
- Mate:112: 3DPRINT,HUB:1 ↔ CAST,SLAB-OF-FLOP:4
- Mate:113: 3DPRINT,HUB:1 ↔ CAST,SLAB-OF-FLOP:4
- Mate:114: 3DPRINT,HUB:1 ↔ CAST,SLAB-OF-FLOP:5
- Insert:142: PLATE,SHOOTER,MOUNT:1 ↔ PURCHASED,10-32x0.625in,BUTTONHEAD,BOLT:52
- Insert:143: PLATE,SHOOTER,MOUNT:1 ↔ PURCHASED,10-32x0.625in,BUTTONHEAD,BOLT:53
- Insert:144: PLATE,SHOOTER,MOUNT:1 ↔ PURCHASED,10-32x0.625in,BUTTONHEAD,BOLT:54
- Insert:145: PLATE,SHOOTER,MOUNT:1 ↔ PURCHASED,10-32x0.625in,BUTTONHEAD,BOLT:55
- Insert:146: PLATE,SHOOTER,MOUNT:1 ↔ PURCHASED,10-32x0.625in,BUTTONHEAD,BOLT:56
- Insert:147: PLATE,SHOOTER,MOUNT:1 ↔ PURCHASED,10-32x0.625in,BUTTONHEAD,BOLT:57
- Mate:117: 3DPRINT,HUB:1 ↔ PLATE,BOTTOM:1
- Mate:118: 3DPRINT,HUB:1 ↔ PLATE,BOTTOM:1
- Mate:119: 3DPRINT,HUB:1 ↔ PLATE,BOTTOM:1
- Flush:24 (-3.175 mm): PLATE,WALL:1 ↔ PLATE,BOTTOM:1
- Mate:120: 3DPRINT,HUB:1 ↔ CAST,SLAB-OF-FLOP:5
- Mate:121: STOCK,HEX,SHAFT,HUB:1 ↔ PURCHASED,20-1,90deg,MAX-PLANETARY:1
- Mate:122 (6.35 mm): PLATE,BOTTOM:1 ↔ PURCHASED,20-1,90deg,MAX-PLANETARY:1
- Insert:148: PURCHASED,20-1,90deg,MAX-PLANETARY:1 ↔ MOTOR,NEO,V2.0:1
- Mate:123: PURCHASED,20-1,90deg,MAX-PLANETARY:1 ↔ MOTOR,NEO,V2.0:1
- Insert:149: 3DPRINT,SPARK_MAX,MOUNT:1 ↔ PLATE,KICKER,BACK:1
- Mate:124: 3DPRINT,SPARK_MAX,MOUNT:1 ↔ PLATE,KICKER,BACK:1
- Mate:125: CONTROLS,SPARK_MAX:1 ↔ PLATE,KICKER,BACK:1
- Mate:126: CONTROLS,SPARK_MAX:1 ↔ 3DPRINT,SPARK_MAX,MOUNT:1
- Mate:127: CONTROLS,SPARK_MAX:1 ↔ 3DPRINT,SPARK_MAX,MOUNT:1
- Mate:128: STOCK,HEX,SHAFT,KICKER,FRONT:1 ↔ PURCHASED,WHEEL,COMPLIANT,2.25in:1
- Mate:129: STOCK,HEX,SHAFT,KICKER,FRONT:1 ↔ PURCHASED,WHEEL,COMPLIANT,2.25in:2
- Mate:130: STOCK,HEX,SHAFT,KICKER,FRONT:1 ↔ PURCHASED,WHEEL,COMPLIANT,2.25in:3
- Mate:131: STOCK,HEX,SHAFT,KICKER,BACK:1 ↔ PURCHASED,WHEEL,COMPLIANT,2.25in:5
- Mate:132: STOCK,HEX,SHAFT,KICKER,BACK:1 ↔ PURCHASED,WHEEL,COMPLIANT,2.25in:6
- Mate:133: STOCK,HEX,SHAFT,KICKER,BACK:1 ↔ PURCHASED,WHEEL,COMPLIANT,2.25in:4
- Mate:134: PURCHASED,WHEEL,COMPLIANT,2.25in:4 ↔ PURCHASED,WHEEL,COMPLIANT,2.25in:5
- Mate:135: PURCHASED,WHEEL,COMPLIANT,2.25in:5 ↔ PURCHASED,WHEEL,COMPLIANT,2.25in:6
- Mate:136: PURCHASED,WHEEL,COMPLIANT,2.25in:1 ↔ PURCHASED,WHEEL,COMPLIANT,2.25in:3
- Mate:137: PURCHASED,WHEEL,COMPLIANT,2.25in:1 ↔ PURCHASED,WHEEL,COMPLIANT,2.25in:2
- Mate:138 (41.275 mm): PLATE,KICKER,OUTSIDE:1 ↔ PURCHASED,WHEEL,COMPLIANT,2.25in:3
- Mate:139 (41.275 mm): PLATE,KICKER,OUTSIDE:1 ↔ PURCHASED,WHEEL,COMPLIANT,2.25in:6
- Insert:150: PLATE,SHOOTER,MOUNT:1 ↔ STOCK,CHURRO,HEX,TURRET,MOTOR-MOUNT,SPACER:1
- Insert:151: PLATE,SHOOTER,MOUNT:1 ↔ STOCK,CHURRO,HEX,TURRET,MOTOR-MOUNT,SPACER:3
- Insert:152: PLATE,SHOOTER,MOUNT:1 ↔ STOCK,CHURRO,HEX,TURRET,MOTOR-MOUNT,SPACER:2
- Insert:153: PLATE,SHOOTER,MOUNT:1 ↔ PURCHASED,HEX_BEARING:7
- Insert:154: PLATE,SHOOTER,MOUNT:1 ↔ PURCHASED,HEX_BEARING:6
- Insert:155: PLATE,TURRET,MOTOR,MOUNT:1 ↔ PURCHASED,HEX_BEARING:8
- Insert:156: PLATE,TURRET,MOTOR,MOUNT:1 ↔ STOCK,CHURRO,HEX,TURRET,MOTOR-MOUNT,SPACER:3
- Insert:157: PLATE,TURRET,MOTOR,MOUNT:1 ↔ STOCK,CHURRO,HEX,TURRET,MOTOR-MOUNT,SPACER:2
- Insert:158: PLATE,SHOOTER,MOUNT:1 ↔ PURCHASED,0.25-20x0.5in,BUTTONHEAD,BOLT:4
- Insert:159: PLATE,SHOOTER,MOUNT:1 ↔ PURCHASED,0.25-20x0.5in,BUTTONHEAD,BOLT:6
- Insert:160: PLATE,SHOOTER,MOUNT:1 ↔ PURCHASED,0.25-20x0.5in,BUTTONHEAD,BOLT:5
- Insert:161: PLATE,TURRET,MOTOR,MOUNT:1 ↔ PURCHASED,0.25-20x0.5in,BUTTONHEAD,BOLT:7
- Insert:162: PLATE,TURRET,MOTOR,MOUNT:1 ↔ PURCHASED,0.25-20x0.5in,BUTTONHEAD,BOLT:8
- Insert:163: PLATE,TURRET,MOTOR,MOUNT:1 ↔ PURCHASED,0.25-20x0.5in,BUTTONHEAD,BOLT:9
- Flush:25: PLATE,TURRET,PINNION,GEAR:1 ↔ STOCK,HEX,SHAFT,TURRET,DRIVE:1
- Mate:140: PLATE,TURRET,PINNION,GEAR:1 ↔ STOCK,HEX,SHAFT,TURRET,DRIVE:1
- Mate:141: PLATE,TURRET,PINNION,GEAR:1 ↔ 3DPRINT,TURRET,HEX,SPACER:2
- Mate:142: STOCK,HEX,SHAFT,TURRET,DRIVE:1 ↔ 3DPRINT,TURRET,HEX,SPACER:2
- Mate:143: PLATE,TURRET,ENCODER,GEAR:1 ↔ STOCK,HEX,SHAFT,TURRET,ENCODER:1
- Flush:26: PLATE,TURRET,ENCODER,GEAR:1 ↔ STOCK,HEX,SHAFT,TURRET,ENCODER:1
- Mate:144: STOCK,HEX,SHAFT,TURRET,ENCODER:1 ↔ 3DPRINT,TURRET,HEX,SPACER:1
- Mate:145: PURCHASED,HEX_BEARING:7 ↔ 3DPRINT,TURRET,HEX,SPACER:1
- Insert:164: PLATE,SHOOTER,MOUNT:1 ↔ STOCK,CHURRO,HEX,TURRET,MOTOR-MOUNT,SPACER:4
- Insert:165: PLATE,SHOOTER,MOUNT:1 ↔ STOCK,CHURRO,HEX,TURRET,MOTOR-MOUNT,SPACER:5
- Insert:166: PLATE,SHOOTER,MOUNT:1 ↔ STOCK,CHURRO,HEX,TURRET,MOTOR-MOUNT,SPACER:6
- Insert:167: PLATE,TURRET,MOTOR,MOUNT:2 ↔ STOCK,CHURRO,HEX,TURRET,MOTOR-MOUNT,SPACER:5
- Mate:146: STOCK,CHURRO,HEX,TURRET,MOTOR-MOUNT,SPACER:4 ↔ PLATE,TURRET,MOTOR,MOUNT:2
- Insert:168: PLATE,SHOOTER,MOUNT:1 ↔ PURCHASED,0.25-20x0.5in,BUTTONHEAD,BOLT:10
- Insert:169: PLATE,SHOOTER,MOUNT:1 ↔ PURCHASED,0.25-20x0.5in,BUTTONHEAD,BOLT:11
- Insert:170: PLATE,SHOOTER,MOUNT:1 ↔ PURCHASED,0.25-20x0.5in,BUTTONHEAD,BOLT:12
- Insert:171: PLATE,TURRET,MOTOR,MOUNT:2 ↔ PURCHASED,0.25-20x0.5in,BUTTONHEAD,BOLT:13
- Insert:172: PLATE,TURRET,MOTOR,MOUNT:2 ↔ PURCHASED,0.25-20x0.5in,BUTTONHEAD,BOLT:14
- Insert:173: PLATE,TURRET,MOTOR,MOUNT:2 ↔ PURCHASED,0.25-20x0.5in,BUTTONHEAD,BOLT:15
- Insert:174: PLATE,TURRET,MOTOR,MOUNT:1 ↔ PURCHASED,10-32x0.625in,BUTTONHEAD,BOLT:61
- Insert:175: PLATE,TURRET,MOTOR,MOUNT:1 ↔ PURCHASED,10-32x0.625in,BUTTONHEAD,BOLT:60
- Insert:176: PLATE,TURRET,MOTOR,MOUNT:1 ↔ PURCHASED,10-32x0.625in,BUTTONHEAD,BOLT:59
- Insert:177: PLATE,TURRET,MOTOR,MOUNT:1 ↔ PURCHASED,10-32x0.625in,BUTTONHEAD,BOLT:58
- Mate:147: PLATE,TURRET,MOTOR,MOUNT:1 ↔ PURCHASED,REV,MAX-PLANETARY,SINGLE-STAGE,FALCON-TO-HEX:1
- Insert:178: PLATE,TURRET,MOTOR,MOUNT:1 ↔ PURCHASED,REV,MAX-PLANETARY,SINGLE-STAGE,FALCON-TO-HEX:1
- Mate:148: PLATE,TURRET,MOTOR,MOUNT:1 ↔ PURCHASED,REV,MAX-PLANETARY,SINGLE-STAGE,FALCON-TO-HEX:1
- Insert:179: MOTOR,VEX,FALCON,500:1 ↔ PURCHASED,REV,MAX-PLANETARY,SINGLE-STAGE,FALCON-TO-HEX:1
- Mate:149: MOTOR,VEX,FALCON,500:1 ↔ PURCHASED,REV,MAX-PLANETARY,SINGLE-STAGE,FALCON-TO-HEX:1
- Insert:180: PLATE,TURRET,MOTOR,MOUNT:2 ↔ PURCHASED,HEX_BEARING:9
- Mate:150: PLATE,SHOOTER,MOUNT:1 ↔ PURCHASED,10-32x0.625in,BUTTONHEAD,BOLT:44
- Mate:151: PLATE,SHOOTER,MOUNT:1 ↔ PURCHASED,10-32x0.625in,BUTTONHEAD,BOLT:46
- Insert:185: PLATE,SHOOTER,MOUNT:1 ↔ PURCHASED,10-32x0.625in,FLATHEAD,BOLT:1
- Insert:186: PLATE,SHOOTER,MOUNT:1 ↔ PURCHASED,10-32x0.625in,FLATHEAD,BOLT:2
- Insert:187: PLATE,SHOOTER,MOUNT:1 ↔ PURCHASED,10-32x0.625in,FLATHEAD,BOLT:3
- Insert:188: PLATE,SHOOTER,MOUNT:1 ↔ PURCHASED,10-32x0.625in,FLATHEAD,BOLT:4
- Insert:210: PLATE,KICKER,INSIDE:1 ↔ PLATE,NUT-BLOCK,3-LONG:4
- Insert:211: PLATE,KICKER,INSIDE:1 ↔ PURCHASED,10-32x0.625in,FLATHEAD,BOLT:5
- Insert:212: PLATE,KICKER,INSIDE:1 ↔ PURCHASED,10-32x0.625in,FLATHEAD,BOLT:6
- Insert:213: PLATE,KICKER,OUTSIDE:1 ↔ PURCHASED,10-32x0.625in,FLATHEAD,BOLT:8
- Insert:214: PLATE,KICKER,OUTSIDE:1 ↔ PURCHASED,10-32x0.625in,FLATHEAD,BOLT:7
- Insert:215: STOCK,HEX,SHAFT,TURRET,DRIVE:1 ↔ PURCHASED,WASHER,10-32:11
- Insert:216: STOCK,HEX,SHAFT,TURRET,ENCODER:1 ↔ PURCHASED,WASHER,10-32:13
- Insert:217: STOCK,HEX,SHAFT,TURRET,ENCODER:1 ↔ PURCHASED,WASHER,10-32:12
- Insert:218: PURCHASED,WASHER,10-32:11 ↔ PURCHASED,10-32x0.625in,BUTTONHEAD,BOLT:62
- Insert:219: PURCHASED,WASHER,10-32:13 ↔ PURCHASED,10-32x0.625in,BUTTONHEAD,BOLT:63
- Insert:220: PURCHASED,WASHER,10-32:12 ↔ PURCHASED,10-32x0.625in,BUTTONHEAD,BOLT:64
- Insert:221: PLATE,SHOOTER,MOUNT:1 ↔ PURCHASED,10-32x0.5in,BUTTONHEAD,BOLT:11
- Insert:222: PLATE,SHOOTER,MOUNT:1 ↔ PURCHASED,10-32x0.5in,BUTTONHEAD,BOLT:12
- Insert:223: PLATE,SHOOTER,MOUNT:1 ↔ PURCHASED,10-32x0.5in,BUTTONHEAD,BOLT:13
- Insert:224: PLATE,SHOOTER,MOUNT:1 ↔ PURCHASED,10-32x0.5in,BUTTONHEAD,BOLT:14
- Insert:225: PLATE,SHOOTER,MOUNT:1 ↔ PURCHASED,10-32x0.5in,BUTTONHEAD,BOLT:15
- Insert:226: PLATE,SHOOTER,MOUNT:1 ↔ PURCHASED,10-32x0.5in,BUTTONHEAD,BOLT:16
- Insert:227: PLATE,SHOOTER,MOUNT:1 ↔ PURCHASED,10-32x0.5in,BUTTONHEAD,BOLT:17
- Insert:228: PLATE,SHOOTER,MOUNT:1 ↔ PURCHASED,10-32x0.5in,BUTTONHEAD,BOLT:18
- Insert:229: PLATE,KICKER,BACK:1 ↔ PURCHASED,10-32x0.625in,BUTTONHEAD,BOLT:65
- Insert:230: PLATE,KICKER,BACK:1 ↔ PURCHASED,10-32x0.625in,BUTTONHEAD,BOLT:66
- Insert:231: PLATE,SHOOTER,MOUNT:1 ↔ PURCHASED,10-32x0.625in,BUTTONHEAD,BOLT:44
- Insert:232: CONTROLS,ENCODER,HEX_BORE:2 ↔ PURCHASED,NYLOCK,10-32,NUT:6
- Insert:233: PLATE,SHOOTER,MOUNT:1 ↔ PURCHASED,10-32x0.625in,BUTTONHEAD,BOLT:45
- Insert:234: CONTROLS,ENCODER,HEX_BORE:2 ↔ PURCHASED,NYLOCK,10-32,NUT:5
- Insert:235: PLATE,SHOOTER,MOUNT:1 ↔ PURCHASED,10-32x0.625in,BUTTONHEAD,BOLT:47
- Insert:236: CONTROLS,ENCODER,HEX_BORE:1 ↔ PURCHASED,NYLOCK,10-32,NUT:8
- Insert:237: PLATE,SHOOTER,MOUNT:1 ↔ PURCHASED,10-32x0.625in,BUTTONHEAD,BOLT:46
- Insert:238: CONTROLS,ENCODER,HEX_BORE:1 ↔ PURCHASED,NYLOCK,10-32,NUT:7
